# Autodesk Inventor assembly: 2nd_Arm_Assembly
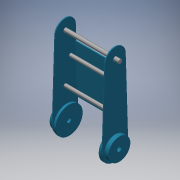
[picture p0: Inventor's stored thumbnail of the model, 180x180]
Saved by Autodesk Inventor 2016 (Build 200138000, 138)
## iProperties
Created: 2015-05-19
Part Number: 2nd_Arm_Assembly
Document SubType Name: Assembly
Designer: CHUNGBK
Author: CHUNGBK
## Documents named in this file (4)
- C:\Users\jonathan\Desktop\Five Axis Serial Robotic Arm\Inventor\Scorbot Shoulder.iam
- C:\Users\jonathan\Desktop\Five Axis Serial Robotic Arm\Inventor\Shoulder.ipt
- C:\Users\jonathan\Desktop\Five Axis Serial Robotic Arm\Inventor\Shoulder Rod.ipt
- C:\Users\jonathan\Desktop\Five Axis Serial Robotic Arm\Inventor\Shoulder Pivot.ipt
## Components (4 placed, 3 different names)
1. Shoulder:1 — Flush:1, Flush:2, Flush:3, Mate:1, Mate:2, Mate:3, Mate:4, Mate:5, Mate:6, Mate:7, Flush:4
2. Shoulder Rod:1 — Mate:4, Mate:5, Mate:6
3. Shoulder Rod:2 — Mate:1, Mate:2, Mate:3
4. Shoulder Pivot:1 — Mate:7, Flush:4
## Relationships (11: Mate 7, Flush 4)
- Flush:1: Shoulder:1
- Flush:2: Shoulder:1
- Flush:3: Shoulder:1
- Mate:1: Shoulder:1 ↔ Shoulder Rod:2
- Mate:2 (-33.3375 mm): Shoulder:1 ↔ Shoulder Rod:2
- Mate:3 (82.55 mm): Shoulder:1 ↔ Shoulder Rod:2
- Mate:4: Shoulder:1 ↔ Shoulder Rod:1
- Mate:5 (-17.4625 mm): Shoulder:1 ↔ Shoulder Rod:1
- Mate:6 (71.4375 mm): Shoulder:1 ↔ Shoulder Rod:1
- Mate:7: Shoulder:1 ↔ Shoulder Pivot:1
- Flush:4 (-13.8748 mm): Shoulder:1 ↔ Shoulder Pivot:1
